# Autodesk Inventor assembly: SupportAssembly
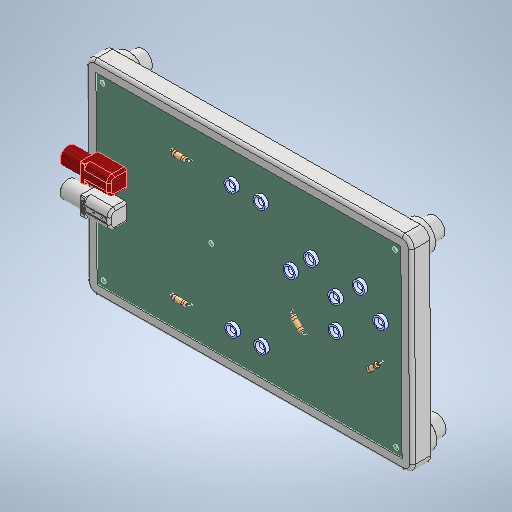
[picture p0: Inventor's stored thumbnail of the model, 512x512]
Saved by Autodesk Inventor 2025 (Build 290162000, 162)
## iProperties
Created: 2026-01-23
Part Number: SupportAssembly
Document SubType Name: Assembly
Designer: tapen
Author: tapen
## Documents named in this file (4)
- C:\Users\tapen\OneDrive\Desktop\Chris Bidinosti\KVL+KCL\SupportFrame\SupportAssembly.iam
- C:\Users\tapen\OneDrive\Desktop\Chris Bidinosti\KVL+KCL\SupportFrame\SupportFrame.ipt
- C:\Users\tapen\OneDrive\Desktop\Chris Bidinosti\KVL+KCL\SupportFrame\KVL+KCL\KVL+KCL.iam
- C:\Users\tapen\OneDrive\Desktop\Chris Bidinosti\KVL+KCL\SupportFrame\rubberFeet.ipt
## Components (6 placed, 3 different names)
1. SupportFrame:1 — Mate:9, Mate:10, Mate:11, Mate:12, Mate:13, Mate:14, Mate:15, Mate:16, Mate:17, Mate:18, Mate:19
2. KVL+KCL:1 [sub-assembly] — Mate:9, Mate:10, Mate:11
3. rubberFeet:1 — Mate:14, Mate:16
4. rubberFeet:2 — Mate:15, Mate:17
5. rubberFeet:3 — Mate:13, Mate:19
6. rubberFeet:4 — Mate:12, Mate:18
## Relationships (11: Mate 11)
- Mate:9: SupportFrame:1 ↔ KVL+KCL:1
- Mate:10: SupportFrame:1 ↔ KVL+KCL:1
- Mate:11: SupportFrame:1 ↔ KVL+KCL:1
- Mate:12: SupportFrame:1 ↔ rubberFeet:4
- Mate:13: SupportFrame:1 ↔ rubberFeet:3
- Mate:14: SupportFrame:1 ↔ rubberFeet:1
- Mate:15: SupportFrame:1 ↔ rubberFeet:2
- Mate:16: SupportFrame:1 ↔ rubberFeet:1
- Mate:17: SupportFrame:1 ↔ rubberFeet:2
- Mate:18: SupportFrame:1 ↔ rubberFeet:4
- Mate:19: SupportFrame:1 ↔ rubberFeet:3
